# Autodesk Inventor assembly: 3.25 Omni AS, cir_MIR2
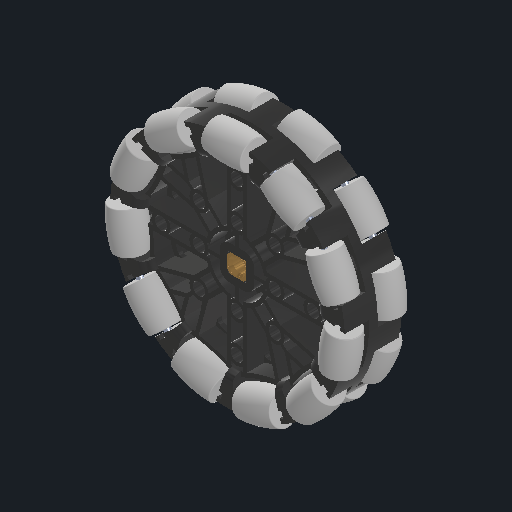
[picture p0: Inventor's stored thumbnail of the model, 512x512]
Saved by Autodesk Inventor 2024 (Build 280153000, 153)
## iProperties
Created: 2023-08-12
Part Number: 3.25 Omni AS, cir_MIR2
Document SubType Name: Assembly
Designer: macbook
Author: macbook
## Documents named in this file (3)
- \\Mac\Home\Desktop\code\1599V-VRC\Cad\Motion\Wheels\Omni Wheel\3.25 Omni AS, cir_MIR2.iam
- \\Mac\Home\Desktop\code\1599V-VRC\Cad\Motion\Wheels\Omni Wheel\3.25 Omni AS, No Insert_MIR2.iam
- \\Mac\Home\Desktop\code\1599V-VRC\Cad\Motion\HS Shaft Adapter Circle_MIR4.ipt
## Components (2 placed, 2 different names)
1. 3.25 Omni AS, No Insert_MIR2:1 [sub-assembly] — Insert:1
2. HS Shaft Adapter Circle_MIR4:1 — Insert:1
## Relationships (1: Insert 1)
- Insert:1: 3.25 Omni AS, No Insert_MIR2:1 ↔ HS Shaft Adapter Circle_MIR4:1
